(part 1 of 3)
# Autodesk Inventor assembly: Frame 1771926384246
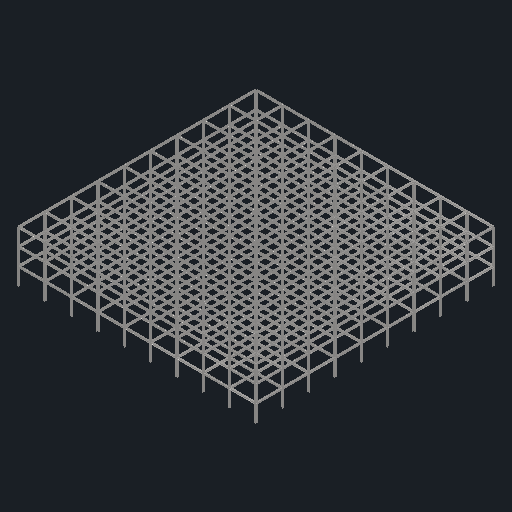
[picture p0: Inventor's stored thumbnail of the model, 512x512]
Saved by Autodesk Inventor 2026.2 (Build 302298010, 298A)
## iProperties
Created: 2026-02-24
Part Number: Frame 1771926384246
Document SubType Name: Assembly
Designer: Admin01
_FrameDoc: Frame Assembly
_Version: 15.0.0
Author: Admin01
## Documents named in this file (842)
- C:\Users\Admin01\Documents\WU15\TRASTRGNN\Inventor\StructureGenerator\Frame\Frame 1771926384246.iam
- C:\Users\Admin01\Documents\WU15\TRASTRGNN\Inventor\StructureGenerator\Frame\Skeleton 1771926384247.ipt
- C:\Users\Admin01\Documents\WU15\TRASTRGNN\Inventor\StructureGenerator\Frame\ANSI UP8 x 30 1771926386924.ipt
- C:\Users\Admin01\Documents\WU15\TRASTRGNN\Inventor\StructureGenerator\Frame\ANSI UP8 x 30 1771926386954.ipt
- C:\Users\Admin01\Documents\WU15\TRASTRGNN\Inventor\StructureGenerator\Frame\ANSI UP8 x 30 1771926386984.ipt
- C:\Users\Admin01\Documents\WU15\TRASTRGNN\Inventor\StructureGenerator\Frame\ANSI UP8 x 30 1771926387014.ipt
- C:\Users\Admin01\Documents\WU15\TRASTRGNN\Inventor\StructureGenerator\Frame\ANSI UP8 x 30 1771926387045.ipt
- C:\Users\Admin01\Documents\WU15\TRASTRGNN\Inventor\StructureGenerator\Frame\ANSI UP8 x 30 1771926387076.ipt
- C:\Users\Admin01\Documents\WU15\TRASTRGNN\Inventor\StructureGenerator\Frame\ANSI UP8 x 30 1771926387107.ipt
- C:\Users\Admin01\Documents\WU15\TRASTRGNN\Inventor\StructureGenerator\Frame\ANSI UP8 x 30 1771926387138.ipt
- C:\Users\Admin01\Documents\WU15\TRASTRGNN\Inventor\StructureGenerator\Frame\ANSI UP8 x 30 1771926387168.ipt
- C:\Users\Admin01\Documents\WU15\TRASTRGNN\Inventor\StructureGenerator\Frame\ANSI UP8 x 30 1771926387199.ipt
- C:\Users\Admin01\Documents\WU15\TRASTRGNN\Inventor\StructureGenerator\Frame\ANSI UP8 x 30 1771926387229.ipt
- C:\Users\Admin01\Documents\WU15\TRASTRGNN\Inventor\StructureGenerator\Frame\ANSI UP8 x 30 1771926387258.ipt
- C:\Users\Admin01\Documents\WU15\TRASTRGNN\Inventor\StructureGenerator\Frame\ANSI UP8 x 30 1771926387288.ipt
- C:\Users\Admin01\Documents\WU15\TRASTRGNN\Inventor\StructureGenerator\Frame\ANSI UP8 x 30 1771926387318.ipt
- C:\Users\Admin01\Documents\WU15\TRASTRGNN\Inventor\StructureGenerator\Frame\ANSI UP8 x 30 1771926387348.ipt
- C:\Users\Admin01\Documents\WU15\TRASTRGNN\Inventor\StructureGenerator\Frame\ANSI UP8 x 30 1771926387378.ipt
- C:\Users\Admin01\Documents\WU15\TRASTRGNN\Inventor\StructureGenerator\Frame\ANSI UP8 x 30 1771926387408.ipt
- C:\Users\Admin01\Documents\WU15\TRASTRGNN\Inventor\StructureGenerator\Frame\ANSI UP8 x 30 1771926387438.ipt
- C:\Users\Admin01\Documents\WU15\TRASTRGNN\Inventor\StructureGenerator\Frame\ANSI UP8 x 30 1771926387467.ipt
- C:\Users\Admin01\Documents\WU15\TRASTRGNN\Inventor\StructureGenerator\Frame\ANSI UP8 x 30 1771926387497.ipt
- C:\Users\Admin01\Documents\WU15\TRASTRGNN\Inventor\StructureGenerator\Frame\ANSI UP8 x 30 1771926387527.ipt
- C:\Users\Admin01\Documents\WU15\TRASTRGNN\Inventor\StructureGenerator\Frame\ANSI UP8 x 30 1771926387557.ipt
- C:\Users\Admin01\Documents\WU15\TRASTRGNN\Inventor\StructureGenerator\Frame\ANSI UP8 x 30 1771926387586.ipt
- C:\Users\Admin01\Documents\WU15\TRASTRGNN\Inventor\StructureGenerator\Frame\ANSI UP8 x 30 1771926387616.ipt
- C:\Users\Admin01\Documents\WU15\TRASTRGNN\Inventor\StructureGenerator\Frame\ANSI UP8 x 30 1771926387646.ipt
- C:\Users\Admin01\Documents\WU15\TRASTRGNN\Inventor\StructureGenerator\Frame\ANSI UP8 x 30 1771926387675.ipt
- C:\Users\Admin01\Documents\WU15\TRASTRGNN\Inventor\StructureGenerator\Frame\ANSI UP8 x 30 1771926387705.ipt
- C:\Users\Admin01\Documents\WU15\TRASTRGNN\Inventor\StructureGenerator\Frame\ANSI UP8 x 30 1771926387735.ipt
- C:\Users\Admin01\Documents\WU15\TRASTRGNN\Inventor\StructureGenerator\Frame\ANSI UP8 x 30 1771926387764.ipt
- C:\Users\Admin01\Documents\WU15\TRASTRGNN\Inventor\StructureGenerator\Frame\ANSI UP8 x 30 1771926387794.ipt
- C:\Users\Admin01\Documents\WU15\TRASTRGNN\Inventor\StructureGenerator\Frame\ANSI UP8 x 30 1771926387824.ipt
- C:\Users\Admin01\Documents\WU15\TRASTRGNN\Inventor\StructureGenerator\Frame\ANSI UP8 x 30 1771926387853.ipt
- C:\Users\Admin01\Documents\WU15\TRASTRGNN\Inventor\StructureGenerator\Frame\ANSI UP8 x 30 1771926387882.ipt
- C:\Users\Admin01\Documents\WU15\TRASTRGNN\Inventor\StructureGenerator\Frame\ANSI UP8 x 30 1771926387912.ipt
- C:\Users\Admin01\Documents\WU15\TRASTRGNN\Inventor\StructureGenerator\Frame\ANSI UP8 x 30 1771926387945.ipt
- C:\Users\Admin01\Documents\WU15\TRASTRGNN\Inventor\StructureGenerator\Frame\ANSI UP8 x 30 1771926387975.ipt
- C:\Users\Admin01\Documents\WU15\TRASTRGNN\Inventor\StructureGenerator\Frame\ANSI UP8 x 30 1771926388005.ipt
- C:\Users\Admin01\Documents\WU15\TRASTRGNN\Inventor\StructureGenerator\Frame\ANSI UP8 x 30 1771926388034.ipt
- C:\Users\Admin01\Documents\WU15\TRASTRGNN\Inventor\StructureGenerator\Frame\ANSI UP8 x 30 1771926388063.ipt
- C:\Users\Admin01\Documents\WU15\TRASTRGNN\Inventor\StructureGenerator\Frame\ANSI UP8 x 30 1771926388093.ipt
- C:\Users\Admin01\Documents\WU15\TRASTRGNN\Inventor\StructureGenerator\Frame\ANSI UP8 x 30 1771926388122.ipt
- C:\Users\Admin01\Documents\WU15\TRASTRGNN\Inventor\StructureGenerator\Frame\ANSI UP8 x 30 1771926388152.ipt
- C:\Users\Admin01\Documents\WU15\TRASTRGNN\Inventor\StructureGenerator\Frame\ANSI UP8 x 30 1771926388182.ipt
- C:\Users\Admin01\Documents\WU15\TRASTRGNN\Inventor\StructureGenerator\Frame\ANSI UP8 x 30 1771926388211.ipt
- C:\Users\Admin01\Documents\WU15\TRASTRGNN\Inventor\StructureGenerator\Frame\ANSI UP8 x 30 1771926388240.ipt
- C:\Users\Admin01\Documents\WU15\TRASTRGNN\Inventor\StructureGenerator\Frame\ANSI UP8 x 30 1771926388269.ipt
- C:\Users\Admin01\Documents\WU15\TRASTRGNN\Inventor\StructureGenerator\Frame\ANSI UP8 x 30 1771926388299.ipt
- C:\Users\Admin01\Documents\WU15\TRASTRGNN\Inventor\StructureGenerator\Frame\ANSI UP8 x 30 1771926388328.ipt
- C:\Users\Admin01\Documents\WU15\TRASTRGNN\Inventor\StructureGenerator\Frame\ANSI UP8 x 30 1771926388357.ipt
- C:\Users\Admin01\Documents\WU15\TRASTRGNN\Inventor\StructureGenerator\Frame\ANSI UP8 x 30 1771926388386.ipt
- C:\Users\Admin01\Documents\WU15\TRASTRGNN\Inventor\StructureGenerator\Frame\ANSI UP8 x 30 1771926388416.ipt
- C:\Users\Admin01\Documents\WU15\TRASTRGNN\Inventor\StructureGenerator\Frame\ANSI UP8 x 30 1771926388446.ipt
- C:\Users\Admin01\Documents\WU15\TRASTRGNN\Inventor\StructureGenerator\Frame\ANSI UP8 x 30 1771926388475.ipt
- C:\Users\Admin01\Documents\WU15\TRASTRGNN\Inventor\StructureGenerator\Frame\ANSI UP8 x 30 1771926388505.ipt
- C:\Users\Admin01\Documents\WU15\TRASTRGNN\Inventor\StructureGenerator\Frame\ANSI UP8 x 30 1771926388535.ipt
- C:\Users\Admin01\Documents\WU15\TRASTRGNN\Inventor\StructureGenerator\Frame\ANSI UP8 x 30 1771926388565.ipt
- C:\Users\Admin01\Documents\WU15\TRASTRGNN\Inventor\StructureGenerator\Frame\ANSI UP8 x 30 1771926388594.ipt
- C:\Users\Admin01\Documents\WU15\TRASTRGNN\Inventor\StructureGenerator\Frame\ANSI UP8 x 30 1771926388624.ipt
- C:\Users\Admin01\Documents\WU15\TRASTRGNN\Inventor\StructureGenerator\Frame\ANSI UP8 x 30 1771926388653.ipt
- C:\Users\Admin01\Documents\WU15\TRASTRGNN\Inventor\StructureGenerator\Frame\ANSI UP8 x 30 1771926388683.ipt
- C:\Users\Admin01\Documents\WU15\TRASTRGNN\Inventor\StructureGenerator\Frame\ANSI UP8 x 30 1771926388713.ipt
- C:\Users\Admin01\Documents\WU15\TRASTRGNN\Inventor\StructureGenerator\Frame\ANSI UP8 x 30 1771926388742.ipt
- C:\Users\Admin01\Documents\WU15\TRASTRGNN\Inventor\StructureGenerator\Frame\ANSI UP8 x 30 1771926388771.ipt
- C:\Users\Admin01\Documents\WU15\TRASTRGNN\Inventor\StructureGenerator\Frame\ANSI UP8 x 30 1771926388800.ipt
- C:\Users\Admin01\Documents\WU15\TRASTRGNN\Inventor\StructureGenerator\Frame\ANSI UP8 x 30 1771926388830.ipt
- C:\Users\Admin01\Documents\WU15\TRASTRGNN\Inventor\StructureGenerator\Frame\ANSI UP8 x 30 1771926388859.ipt
- C:\Users\Admin01\Documents\WU15\TRASTRGNN\Inventor\StructureGenerator\Frame\ANSI UP8 x 30 1771926388888.ipt
- C:\Users\Admin01\Documents\WU15\TRASTRGNN\Inventor\StructureGenerator\Frame\ANSI UP8 x 30 1771926388918.ipt
- C:\Users\Admin01\Documents\WU15\TRASTRGNN\Inventor\StructureGenerator\Frame\ANSI UP8 x 30 1771926388947.ipt
- C:\Users\Admin01\Documents\WU15\TRASTRGNN\Inventor\StructureGenerator\Frame\ANSI UP8 x 30 1771926388977.ipt
- C:\Users\Admin01\Documents\WU15\TRASTRGNN\Inventor\StructureGenerator\Frame\ANSI UP8 x 30 1771926389006.ipt
- C:\Users\Admin01\Documents\WU15\TRASTRGNN\Inventor\StructureGenerator\Frame\ANSI UP8 x 30 1771926389039.ipt
- C:\Users\Admin01\Documents\WU15\TRASTRGNN\Inventor\StructureGenerator\Frame\ANSI UP8 x 30 1771926389068.ipt
- C:\Users\Admin01\Documents\WU15\TRASTRGNN\Inventor\StructureGenerator\Frame\ANSI UP8 x 30 1771926389098.ipt
- C:\Users\Admin01\Documents\WU15\TRASTRGNN\Inventor\StructureGenerator\Frame\ANSI UP8 x 30 1771926389128.ipt
- C:\Users\Admin01\Documents\WU15\TRASTRGNN\Inventor\StructureGenerator\Frame\ANSI UP8 x 30 1771926389158.ipt
- C:\Users\Admin01\Documents\WU15\TRASTRGNN\Inventor\StructureGenerator\Frame\ANSI UP8 x 30 1771926389187.ipt
- C:\Users\Admin01\Documents\WU15\TRASTRGNN\Inventor\StructureGenerator\Frame\ANSI UP8 x 30 1771926389216.ipt
- C:\Users\Admin01\Documents\WU15\TRASTRGNN\Inventor\StructureGenerator\Frame\ANSI UP8 x 30 1771926389245.ipt
- C:\Users\Admin01\Documents\WU15\TRASTRGNN\Inventor\StructureGenerator\Frame\ANSI UP8 x 30 1771926389274.ipt
- C:\Users\Admin01\Documents\WU15\TRASTRGNN\Inventor\StructureGenerator\Frame\ANSI UP8 x 30 1771926389303.ipt
- C:\Users\Admin01\Documents\WU15\TRASTRGNN\Inventor\StructureGenerator\Frame\ANSI UP8 x 30 1771926389333.ipt
- C:\Users\Admin01\Documents\WU15\TRASTRGNN\Inventor\StructureGenerator\Frame\ANSI UP8 x 30 1771926389362.ipt
- C:\Users\Admin01\Documents\WU15\TRASTRGNN\Inventor\StructureGenerator\Frame\ANSI UP8 x 30 1771926389391.ipt
- C:\Users\Admin01\Documents\WU15\TRASTRGNN\Inventor\StructureGenerator\Frame\ANSI UP8 x 30 1771926389420.ipt
- C:\Users\Admin01\Documents\WU15\TRASTRGNN\Inventor\StructureGenerator\Frame\ANSI UP8 x 30 1771926389450.ipt
- C:\Users\Admin01\Documents\WU15\TRASTRGNN\Inventor\StructureGenerator\Frame\ANSI UP8 x 30 1771926389479.ipt
- C:\Users\Admin01\Documents\WU15\TRASTRGNN\Inventor\StructureGenerator\Frame\ANSI UP8 x 30 1771926389515.ipt
- C:\Users\Admin01\Documents\WU15\TRASTRGNN\Inventor\StructureGenerator\Frame\ANSI UP8 x 30 1771926389551.ipt
- C:\Users\Admin01\Documents\WU15\TRASTRGNN\Inventor\StructureGenerator\Frame\ANSI UP8 x 30 1771926389587.ipt
- C:\Users\Admin01\Documents\WU15\TRASTRGNN\Inventor\StructureGenerator\Frame\ANSI UP8 x 30 1771926389625.ipt
- C:\Users\Admin01\Documents\WU15\TRASTRGNN\Inventor\StructureGenerator\Frame\ANSI UP8 x 30 1771926389656.ipt
- C:\Users\Admin01\Documents\WU15\TRASTRGNN\Inventor\StructureGenerator\Frame\ANSI UP8 x 30 1771926389685.ipt
- C:\Users\Admin01\Documents\WU15\TRASTRGNN\Inventor\StructureGenerator\Frame\ANSI UP8 x 30 1771926389715.ipt
- C:\Users\Admin01\Documents\WU15\TRASTRGNN\Inventor\StructureGenerator\Frame\ANSI UP8 x 30 1771926389744.ipt
- C:\Users\Admin01\Documents\WU15\TRASTRGNN\Inventor\StructureGenerator\Frame\ANSI UP8 x 30 1771926389773.ipt
- C:\Users\Admin01\Documents\WU15\TRASTRGNN\Inventor\StructureGenerator\Frame\ANSI UP8 x 30 1771926389802.ipt
- C:\Users\Admin01\Documents\WU15\TRASTRGNN\Inventor\StructureGenerator\Frame\ANSI UP8 x 30 1771926389831.ipt
- C:\Users\Admin01\Documents\WU15\TRASTRGNN\Inventor\StructureGenerator\Frame\ANSI UP8 x 30 1771926389860.ipt
- C:\Users\Admin01\Documents\WU15\TRASTRGNN\Inventor\StructureGenerator\Frame\ANSI UP8 x 30 1771926389889.ipt
- C:\Users\Admin01\Documents\WU15\TRASTRGNN\Inventor\StructureGenerator\Frame\ANSI UP8 x 30 1771926389918.ipt
- C:\Users\Admin01\Documents\WU15\TRASTRGNN\Inventor\StructureGenerator\Frame\ANSI UP8 x 30 1771926389947.ipt
- C:\Users\Admin01\Documents\WU15\TRASTRGNN\Inventor\StructureGenerator\Frame\ANSI UP8 x 30 1771926389976.ipt
- C:\Users\Admin01\Documents\WU15\TRASTRGNN\Inventor\StructureGenerator\Frame\ANSI UP8 x 30 1771926390006.ipt
- C:\Users\Admin01\Documents\WU15\TRASTRGNN\Inventor\StructureGenerator\Frame\ANSI UP8 x 30 1771926390034.ipt
- C:\Users\Admin01\Documents\WU15\TRASTRGNN\Inventor\StructureGenerator\Frame\ANSI UP8 x 30 1771926390064.ipt
- C:\Users\Admin01\Documents\WU15\TRASTRGNN\Inventor\StructureGenerator\Frame\ANSI UP8 x 30 1771926390093.ipt
- C:\Users\Admin01\Documents\WU15\TRASTRGNN\Inventor\StructureGenerator\Frame\ANSI UP8 x 30 1771926390122.ipt
- C:\Users\Admin01\Documents\WU15\TRASTRGNN\Inventor\StructureGenerator\Frame\ANSI UP8 x 30 1771926390154.ipt
- C:\Users\Admin01\Documents\WU15\TRASTRGNN\Inventor\StructureGenerator\Frame\ANSI UP8 x 30 1771926390184.ipt
- C:\Users\Admin01\Documents\WU15\TRASTRGNN\Inventor\StructureGenerator\Frame\ANSI UP8 x 30 1771926390213.ipt
- C:\Users\Admin01\Documents\WU15\TRASTRGNN\Inventor\StructureGenerator\Frame\ANSI UP8 x 30 1771926390246.ipt
- C:\Users\Admin01\Documents\WU15\TRASTRGNN\Inventor\StructureGenerator\Frame\ANSI UP8 x 30 1771926390275.ipt
- C:\Users\Admin01\Documents\WU15\TRASTRGNN\Inventor\StructureGenerator\Frame\ANSI UP8 x 30 1771926390304.ipt
- C:\Users\Admin01\Documents\WU15\TRASTRGNN\Inventor\StructureGenerator\Frame\ANSI UP8 x 30 1771926390333.ipt
- C:\Users\Admin01\Documents\WU15\TRASTRGNN\Inventor\StructureGenerator\Frame\ANSI UP8 x 30 1771926390362.ipt
- C:\Users\Admin01\Documents\WU15\TRASTRGNN\Inventor\StructureGenerator\Frame\ANSI UP8 x 30 1771926390391.ipt
- C:\Users\Admin01\Documents\WU15\TRASTRGNN\Inventor\StructureGenerator\Frame\ANSI UP8 x 30 1771926390421.ipt
- C:\Users\Admin01\Documents\WU15\TRASTRGNN\Inventor\StructureGenerator\Frame\ANSI UP8 x 30 1771926390450.ipt
- C:\Users\Admin01\Documents\WU15\TRASTRGNN\Inventor\StructureGenerator\Frame\ANSI UP8 x 30 1771926390480.ipt
- C:\Users\Admin01\Documents\WU15\TRASTRGNN\Inventor\StructureGenerator\Frame\ANSI UP8 x 30 1771926390509.ipt
- C:\Users\Admin01\Documents\WU15\TRASTRGNN\Inventor\StructureGenerator\Frame\ANSI UP8 x 30 1771926390539.ipt
- C:\Users\Admin01\Documents\WU15\TRASTRGNN\Inventor\StructureGenerator\Frame\ANSI UP8 x 30 1771926390569.ipt
- C:\Users\Admin01\Documents\WU15\TRASTRGNN\Inventor\StructureGenerator\Frame\ANSI UP8 x 30 1771926390598.ipt
- C:\Users\Admin01\Documents\WU15\TRASTRGNN\Inventor\StructureGenerator\Frame\ANSI UP8 x 30 1771926390628.ipt
- C:\Users\Admin01\Documents\WU15\TRASTRGNN\Inventor\StructureGenerator\Frame\ANSI UP8 x 30 1771926390658.ipt
- C:\Users\Admin01\Documents\WU15\TRASTRGNN\Inventor\StructureGenerator\Frame\ANSI UP8 x 30 1771926390687.ipt
- C:\Users\Admin01\Documents\WU15\TRASTRGNN\Inventor\StructureGenerator\Frame\ANSI UP8 x 30 1771926390716.ipt
- C:\Users\Admin01\Documents\WU15\TRASTRGNN\Inventor\StructureGenerator\Frame\ANSI UP8 x 30 1771926390746.ipt
- C:\Users\Admin01\Documents\WU15\TRASTRGNN\Inventor\StructureGenerator\Frame\ANSI UP8 x 30 1771926390776.ipt
- C:\Users\Admin01\Documents\WU15\TRASTRGNN\Inventor\StructureGenerator\Frame\ANSI UP8 x 30 1771926390806.ipt
- C:\Users\Admin01\Documents\WU15\TRASTRGNN\Inventor\StructureGenerator\Frame\ANSI UP8 x 30 1771926390836.ipt
- C:\Users\Admin01\Documents\WU15\TRASTRGNN\Inventor\StructureGenerator\Frame\ANSI UP8 x 30 1771926390865.ipt
- C:\Users\Admin01\Documents\WU15\TRASTRGNN\Inventor\StructureGenerator\Frame\ANSI UP8 x 30 1771926390894.ipt
- C:\Users\Admin01\Documents\WU15\TRASTRGNN\Inventor\StructureGenerator\Frame\ANSI UP8 x 30 1771926390924.ipt
- C:\Users\Admin01\Documents\WU15\TRASTRGNN\Inventor\StructureGenerator\Frame\ANSI UP8 x 30 1771926390953.ipt
- C:\Users\Admin01\Documents\WU15\TRASTRGNN\Inventor\StructureGenerator\Frame\ANSI UP8 x 30 1771926390983.ipt
- C:\Users\Admin01\Documents\WU15\TRASTRGNN\Inventor\StructureGenerator\Frame\ANSI UP8 x 30 1771926391012.ipt
- C:\Users\Admin01\Documents\WU15\TRASTRGNN\Inventor\StructureGenerator\Frame\ANSI UP8 x 30 1771926391042.ipt
- C:\Users\Admin01\Documents\WU15\TRASTRGNN\Inventor\StructureGenerator\Frame\ANSI UP8 x 30 1771926391071.ipt
- C:\Users\Admin01\Documents\WU15\TRASTRGNN\Inventor\StructureGenerator\Frame\ANSI UP8 x 30 1771926391102.ipt
- C:\Users\Admin01\Documents\WU15\TRASTRGNN\Inventor\StructureGenerator\Frame\ANSI UP8 x 30 1771926391131.ipt
- C:\Users\Admin01\Documents\WU15\TRASTRGNN\Inventor\StructureGenerator\Frame\ANSI UP8 x 30 1771926391160.ipt
- C:\Users\Admin01\Documents\WU15\TRASTRGNN\Inventor\StructureGenerator\Frame\ANSI UP8 x 30 1771926391190.ipt
- C:\Users\Admin01\Documents\WU15\TRASTRGNN\Inventor\StructureGenerator\Frame\ANSI UP8 x 30 1771926391219.ipt
- C:\Users\Admin01\Documents\WU15\TRASTRGNN\Inventor\StructureGenerator\Frame\ANSI UP8 x 30 1771926391252.ipt
- C:\Users\Admin01\Documents\WU15\TRASTRGNN\Inventor\StructureGenerator\Frame\ANSI UP8 x 30 1771926391282.ipt
- C:\Users\Admin01\Documents\WU15\TRASTRGNN\Inventor\StructureGenerator\Frame\ANSI UP8 x 30 1771926391311.ipt
- C:\Users\Admin01\Documents\WU15\TRASTRGNN\Inventor\StructureGenerator\Frame\ANSI UP8 x 30 1771926391340.ipt
- C:\Users\Admin01\Documents\WU15\TRASTRGNN\Inventor\StructureGenerator\Frame\ANSI UP8 x 30 1771926391369.ipt
- C:\Users\Admin01\Documents\WU15\TRASTRGNN\Inventor\StructureGenerator\Frame\ANSI UP8 x 30 1771926391399.ipt
- C:\Users\Admin01\Documents\WU15\TRASTRGNN\Inventor\StructureGenerator\Frame\ANSI UP8 x 30 1771926391428.ipt
- C:\Users\Admin01\Documents\WU15\TRASTRGNN\Inventor\StructureGenerator\Frame\ANSI UP8 x 30 1771926391457.ipt
- C:\Users\Admin01\Documents\WU15\TRASTRGNN\Inventor\StructureGenerator\Frame\ANSI UP8 x 30 1771926391486.ipt
- C:\Users\Admin01\Documents\WU15\TRASTRGNN\Inventor\StructureGenerator\Frame\ANSI UP8 x 30 1771926391515.ipt
- C:\Users\Admin01\Documents\WU15\TRASTRGNN\Inventor\StructureGenerator\Frame\ANSI UP8 x 30 1771926391549.ipt
- C:\Users\Admin01\Documents\WU15\TRASTRGNN\Inventor\StructureGenerator\Frame\ANSI UP8 x 30 1771926391578.ipt
- C:\Users\Admin01\Documents\WU15\TRASTRGNN\Inventor\StructureGenerator\Frame\ANSI UP8 x 30 1771926391608.ipt
- C:\Users\Admin01\Documents\WU15\TRASTRGNN\Inventor\StructureGenerator\Frame\ANSI UP8 x 30 1771926391637.ipt
- C:\Users\Admin01\Documents\WU15\TRASTRGNN\Inventor\StructureGenerator\Frame\ANSI UP8 x 30 1771926391667.ipt
- C:\Users\Admin01\Documents\WU15\TRASTRGNN\Inventor\StructureGenerator\Frame\ANSI UP8 x 30 1771926391696.ipt
- C:\Users\Admin01\Documents\WU15\TRASTRGNN\Inventor\StructureGenerator\Frame\ANSI UP8 x 30 1771926391725.ipt
- C:\Users\Admin01\Documents\WU15\TRASTRGNN\Inventor\StructureGenerator\Frame\ANSI UP8 x 30 1771926391754.ipt
- C:\Users\Admin01\Documents\WU15\TRASTRGNN\Inventor\StructureGenerator\Frame\ANSI UP8 x 30 1771926391784.ipt
- C:\Users\Admin01\Documents\WU15\TRASTRGNN\Inventor\StructureGenerator\Frame\ANSI UP8 x 30 1771926391813.ipt
- C:\Users\Admin01\Documents\WU15\TRASTRGNN\Inventor\StructureGenerator\Frame\ANSI UP8 x 30 1771926391842.ipt
- C:\Users\Admin01\Documents\WU15\TRASTRGNN\Inventor\StructureGenerator\Frame\ANSI UP8 x 30 1771926391871.ipt
- C:\Users\Admin01\Documents\WU15\TRASTRGNN\Inventor\StructureGenerator\Frame\ANSI UP8 x 30 1771926391900.ipt
- C:\Users\Admin01\Documents\WU15\TRASTRGNN\Inventor\StructureGenerator\Frame\ANSI UP8 x 30 1771926391930.ipt
- C:\Users\Admin01\Documents\WU15\TRASTRGNN\Inventor\StructureGenerator\Frame\ANSI UP8 x 30 1771926391960.ipt
- C:\Users\Admin01\Documents\WU15\TRASTRGNN\Inventor\StructureGenerator\Frame\ANSI UP8 x 30 1771926391990.ipt
- C:\Users\Admin01\Documents\WU15\TRASTRGNN\Inventor\StructureGenerator\Frame\ANSI UP8 x 30 1771926392019.ipt
- C:\Users\Admin01\Documents\WU15\TRASTRGNN\Inventor\StructureGenerator\Frame\ANSI UP8 x 30 1771926392048.ipt
- C:\Users\Admin01\Documents\WU15\TRASTRGNN\Inventor\StructureGenerator\Frame\ANSI UP8 x 30 1771926392077.ipt
- C:\Users\Admin01\Documents\WU15\TRASTRGNN\Inventor\StructureGenerator\Frame\ANSI UP8 x 30 1771926392107.ipt
- C:\Users\Admin01\Documents\WU15\TRASTRGNN\Inventor\StructureGenerator\Frame\ANSI UP8 x 30 1771926392136.ipt
- C:\Users\Admin01\Documents\WU15\TRASTRGNN\Inventor\StructureGenerator\Frame\ANSI UP8 x 30 1771926392166.ipt
- C:\Users\Admin01\Documents\WU15\TRASTRGNN\Inventor\StructureGenerator\Frame\ANSI UP8 x 30 1771926392195.ipt
- C:\Users\Admin01\Documents\WU15\TRASTRGNN\Inventor\StructureGenerator\Frame\ANSI UP8 x 30 1771926392224.ipt
- C:\Users\Admin01\Documents\WU15\TRASTRGNN\Inventor\StructureGenerator\Frame\ANSI UP8 x 30 1771926392253.ipt
- C:\Users\Admin01\Documents\WU15\TRASTRGNN\Inventor\StructureGenerator\Frame\ANSI UP8 x 30 1771926392282.ipt
- C:\Users\Admin01\Documents\WU15\TRASTRGNN\Inventor\StructureGenerator\Frame\ANSI UP8 x 30 1771926392311.ipt
- C:\Users\Admin01\Documents\WU15\TRASTRGNN\Inventor\StructureGenerator\Frame\ANSI UP8 x 30 1771926392344.ipt
- C:\Users\Admin01\Documents\WU15\TRASTRGNN\Inventor\StructureGenerator\Frame\ANSI UP8 x 30 1771926392373.ipt
- C:\Users\Admin01\Documents\WU15\TRASTRGNN\Inventor\StructureGenerator\Frame\ANSI UP8 x 30 1771926392402.ipt
- C:\Users\Admin01\Documents\WU15\TRASTRGNN\Inventor\StructureGenerator\Frame\ANSI UP8 x 30 1771926392432.ipt
- C:\Users\Admin01\Documents\WU15\TRASTRGNN\Inventor\StructureGenerator\Frame\ANSI UP8 x 30 1771926392461.ipt
- C:\Users\Admin01\Documents\WU15\TRASTRGNN\Inventor\StructureGenerator\Frame\ANSI UP8 x 30 1771926392490.ipt
- C:\Users\Admin01\Documents\WU15\TRASTRGNN\Inventor\StructureGenerator\Frame\ANSI UP8 x 30 1771926392520.ipt
- C:\Users\Admin01\Documents\WU15\TRASTRGNN\Inventor\StructureGenerator\Frame\ANSI UP8 x 30 1771926392549.ipt
- C:\Users\Admin01\Documents\WU15\TRASTRGNN\Inventor\StructureGenerator\Frame\ANSI UP8 x 30 1771926392578.ipt
- C:\Users\Admin01\Documents\WU15\TRASTRGNN\Inventor\StructureGenerator\Frame\ANSI UP8 x 30 1771926392607.ipt
- C:\Users\Admin01\Documents\WU15\TRASTRGNN\Inventor\StructureGenerator\Frame\ANSI UP8 x 30 1771926392637.ipt
- C:\Users\Admin01\Documents\WU15\TRASTRGNN\Inventor\StructureGenerator\Frame\ANSI UP8 x 30 1771926392667.ipt
- C:\Users\Admin01\Documents\WU15\TRASTRGNN\Inventor\StructureGenerator\Frame\ANSI UP8 x 30 1771926392696.ipt
- C:\Users\Admin01\Documents\WU15\TRASTRGNN\Inventor\StructureGenerator\Frame\ANSI UP8 x 30 1771926392725.ipt
- C:\Users\Admin01\Documents\WU15\TRASTRGNN\Inventor\StructureGenerator\Frame\ANSI UP8 x 30 1771926392755.ipt
- C:\Users\Admin01\Documents\WU15\TRASTRGNN\Inventor\StructureGenerator\Frame\ANSI UP8 x 30 1771926392784.ipt
- C:\Users\Admin01\Documents\WU15\TRASTRGNN\Inventor\StructureGenerator\Frame\ANSI UP8 x 30 1771926392813.ipt
- C:\Users\Admin01\Documents\WU15\TRASTRGNN\Inventor\StructureGenerator\Frame\ANSI UP8 x 30 1771926392842.ipt
- C:\Users\Admin01\Documents\WU15\TRASTRGNN\Inventor\StructureGenerator\Frame\ANSI UP8 x 30 1771926392872.ipt
- C:\Users\Admin01\Documents\WU15\TRASTRGNN\Inventor\StructureGenerator\Frame\ANSI UP8 x 30 1771926392901.ipt
- C:\Users\Admin01\Documents\WU15\TRASTRGNN\Inventor\StructureGenerator\Frame\ANSI UP8 x 30 1771926392930.ipt
- C:\Users\Admin01\Documents\WU15\TRASTRGNN\Inventor\StructureGenerator\Frame\ANSI UP8 x 30 1771926392960.ipt
- C:\Users\Admin01\Documents\WU15\TRASTRGNN\Inventor\StructureGenerator\Frame\ANSI UP8 x 30 1771926392989.ipt
- C:\Users\Admin01\Documents\WU15\TRASTRGNN\Inventor\StructureGenerator\Frame\ANSI UP8 x 30 1771926393018.ipt
- C:\Users\Admin01\Documents\WU15\TRASTRGNN\Inventor\StructureGenerator\Frame\ANSI UP8 x 30 1771926393048.ipt
- C:\Users\Admin01\Documents\WU15\TRASTRGNN\Inventor\StructureGenerator\Frame\ANSI UP8 x 30 1771926393077.ipt
- C:\Users\Admin01\Documents\WU15\TRASTRGNN\Inventor\StructureGenerator\Frame\ANSI UP8 x 30 1771926393106.ipt
- C:\Users\Admin01\Documents\WU15\TRASTRGNN\Inventor\StructureGenerator\Frame\ANSI UP8 x 30 1771926393136.ipt
- C:\Users\Admin01\Documents\WU15\TRASTRGNN\Inventor\StructureGenerator\Frame\ANSI UP8 x 30 1771926393166.ipt
- C:\Users\Admin01\Documents\WU15\TRASTRGNN\Inventor\StructureGenerator\Frame\ANSI UP8 x 30 1771926393196.ipt
- C:\Users\Admin01\Documents\WU15\TRASTRGNN\Inventor\StructureGenerator\Frame\ANSI UP8 x 30 1771926393225.ipt
- C:\Users\Admin01\Documents\WU15\TRASTRGNN\Inventor\StructureGenerator\Frame\ANSI UP8 x 30 1771926393255.ipt
- C:\Users\Admin01\Documents\WU15\TRASTRGNN\Inventor\StructureGenerator\Frame\ANSI UP8 x 30 1771926393284.ipt
- C:\Users\Admin01\Documents\WU15\TRASTRGNN\Inventor\StructureGenerator\Frame\ANSI UP8 x 30 1771926393313.ipt
- C:\Users\Admin01\Documents\WU15\TRASTRGNN\Inventor\StructureGenerator\Frame\ANSI UP8 x 30 1771926393342.ipt
- C:\Users\Admin01\Documents\WU15\TRASTRGNN\Inventor\StructureGenerator\Frame\ANSI UP8 x 30 1771926393371.ipt
- C:\Users\Admin01\Documents\WU15\TRASTRGNN\Inventor\StructureGenerator\Frame\ANSI UP8 x 30 1771926393400.ipt
- C:\Users\Admin01\Documents\WU15\TRASTRGNN\Inventor\StructureGenerator\Frame\ANSI UP8 x 30 1771926393451.ipt
- C:\Users\Admin01\Documents\WU15\TRASTRGNN\Inventor\StructureGenerator\Frame\ANSI UP8 x 30 1771926393482.ipt
- C:\Users\Admin01\Documents\WU15\TRASTRGNN\Inventor\StructureGenerator\Frame\ANSI UP8 x 30 1771926393513.ipt
- C:\Users\Admin01\Documents\WU15\TRASTRGNN\Inventor\StructureGenerator\Frame\ANSI UP8 x 30 1771926393543.ipt
- C:\Users\Admin01\Documents\WU15\TRASTRGNN\Inventor\StructureGenerator\Frame\ANSI UP8 x 30 1771926393573.ipt
- C:\Users\Admin01\Documents\WU15\TRASTRGNN\Inventor\StructureGenerator\Frame\ANSI UP8 x 30 1771926393603.ipt
- C:\Users\Admin01\Documents\WU15\TRASTRGNN\Inventor\StructureGenerator\Frame\ANSI UP8 x 30 1771926393633.ipt
- C:\Users\Admin01\Documents\WU15\TRASTRGNN\Inventor\StructureGenerator\Frame\ANSI UP8 x 30 1771926393663.ipt
- C:\Users\Admin01\Documents\WU15\TRASTRGNN\Inventor\StructureGenerator\Frame\ANSI UP8 x 30 1771926393693.ipt
- C:\Users\Admin01\Documents\WU15\TRASTRGNN\Inventor\StructureGenerator\Frame\ANSI UP8 x 30 1771926393723.ipt
- C:\Users\Admin01\Documents\WU15\TRASTRGNN\Inventor\StructureGenerator\Frame\ANSI UP8 x 30 1771926393758.ipt
- C:\Users\Admin01\Documents\WU15\TRASTRGNN\Inventor\StructureGenerator\Frame\ANSI UP8 x 30 1771926393788.ipt
- C:\Users\Admin01\Documents\WU15\TRASTRGNN\Inventor\StructureGenerator\Frame\ANSI UP8 x 30 1771926393817.ipt
- C:\Users\Admin01\Documents\WU15\TRASTRGNN\Inventor\StructureGenerator\Frame\ANSI UP8 x 30 1771926393846.ipt
- C:\Users\Admin01\Documents\WU15\TRASTRGNN\Inventor\StructureGenerator\Frame\ANSI UP8 x 30 1771926393875.ipt
- C:\Users\Admin01\Documents\WU15\TRASTRGNN\Inventor\StructureGenerator\Frame\ANSI UP8 x 30 1771926393904.ipt
- C:\Users\Admin01\Documents\WU15\TRASTRGNN\Inventor\StructureGenerator\Frame\ANSI UP8 x 30 1771926393933.ipt
- C:\Users\Admin01\Documents\WU15\TRASTRGNN\Inventor\StructureGenerator\Frame\ANSI UP8 x 30 1771926393963.ipt
- C:\Users\Admin01\Documents\WU15\TRASTRGNN\Inventor\StructureGenerator\Frame\ANSI UP8 x 30 1771926393992.ipt
- C:\Users\Admin01\Documents\WU15\TRASTRGNN\Inventor\StructureGenerator\Frame\ANSI UP8 x 30 1771926394021.ipt
- C:\Users\Admin01\Documents\WU15\TRASTRGNN\Inventor\StructureGenerator\Frame\ANSI UP8 x 30 1771926394050.ipt
- C:\Users\Admin01\Documents\WU15\TRASTRGNN\Inventor\StructureGenerator\Frame\ANSI UP8 x 30 1771926394079.ipt
- C:\Users\Admin01\Documents\WU15\TRASTRGNN\Inventor\StructureGenerator\Frame\ANSI UP8 x 30 1771926394108.ipt
- C:\Users\Admin01\Documents\WU15\TRASTRGNN\Inventor\StructureGenerator\Frame\ANSI UP8 x 30 1771926394137.ipt
- C:\Users\Admin01\Documents\WU15\TRASTRGNN\Inventor\StructureGenerator\Frame\ANSI UP8 x 30 1771926394169.ipt
- C:\Users\Admin01\Documents\WU15\TRASTRGNN\Inventor\StructureGenerator\Frame\ANSI UP8 x 30 1771926394198.ipt
- C:\Users\Admin01\Documents\WU15\TRASTRGNN\Inventor\StructureGenerator\Frame\ANSI UP8 x 30 1771926394228.ipt
- C:\Users\Admin01\Documents\WU15\TRASTRGNN\Inventor\StructureGenerator\Frame\ANSI UP8 x 30 1771926394257.ipt
- C:\Users\Admin01\Documents\WU15\TRASTRGNN\Inventor\StructureGenerator\Frame\ANSI UP8 x 30 1771926394286.ipt
- C:\Users\Admin01\Documents\WU15\TRASTRGNN\Inventor\StructureGenerator\Frame\ANSI UP8 x 30 1771926394316.ipt
- C:\Users\Admin01\Documents\WU15\TRASTRGNN\Inventor\StructureGenerator\Frame\ANSI UP8 x 30 1771926394345.ipt
- C:\Users\Admin01\Documents\WU15\TRASTRGNN\Inventor\StructureGenerator\Frame\ANSI UP8 x 30 1771926394374.ipt
- C:\Users\Admin01\Documents\WU15\TRASTRGNN\Inventor\StructureGenerator\Frame\ANSI UP8 x 30 1771926394404.ipt
- C:\Users\Admin01\Documents\WU15\TRASTRGNN\Inventor\StructureGenerator\Frame\ANSI UP8 x 30 1771926394433.ipt
- C:\Users\Admin01\Documents\WU15\TRASTRGNN\Inventor\StructureGenerator\Frame\ANSI UP8 x 30 1771926394462.ipt
- C:\Users\Admin01\Documents\WU15\TRASTRGNN\Inventor\StructureGenerator\Frame\ANSI UP8 x 30 1771926394492.ipt
- C:\Users\Admin01\Documents\WU15\TRASTRGNN\Inventor\StructureGenerator\Frame\ANSI UP8 x 30 1771926394521.ipt
- C:\Users\Admin01\Documents\WU15\TRASTRGNN\Inventor\StructureGenerator\Frame\ANSI UP8 x 30 1771926394553.ipt
- C:\Users\Admin01\Documents\WU15\TRASTRGNN\Inventor\StructureGenerator\Frame\ANSI UP8 x 30 1771926394582.ipt
- C:\Users\Admin01\Documents\WU15\TRASTRGNN\Inventor\StructureGenerator\Frame\ANSI UP8 x 30 1771926394611.ipt
- C:\Users\Admin01\Documents\WU15\TRASTRGNN\Inventor\StructureGenerator\Frame\ANSI UP8 x 30 1771926394640.ipt
- C:\Users\Admin01\Documents\WU15\TRASTRGNN\Inventor\StructureGenerator\Frame\ANSI UP8 x 30 1771926394669.ipt
- C:\Users\Admin01\Documents\WU15\TRASTRGNN\Inventor\StructureGenerator\Frame\ANSI UP8 x 30 1771926394699.ipt
- C:\Users\Admin01\Documents\WU15\TRASTRGNN\Inventor\StructureGenerator\Frame\ANSI UP8 x 30 1771926394728.ipt
- C:\Users\Admin01\Documents\WU15\TRASTRGNN\Inventor\StructureGenerator\Frame\ANSI UP8 x 30 1771926394757.ipt
- C:\Users\Admin01\Documents\WU15\TRASTRGNN\Inventor\StructureGenerator\Frame\ANSI UP8 x 30 1771926394786.ipt
- C:\Users\Admin01\Documents\WU15\TRASTRGNN\Inventor\StructureGenerator\Frame\ANSI UP8 x 30 1771926394815.ipt
- C:\Users\Admin01\Documents\WU15\TRASTRGNN\Inventor\StructureGenerator\Frame\ANSI UP8 x 30 1771926394844.ipt
- C:\Users\Admin01\Documents\WU15\TRASTRGNN\Inventor\StructureGenerator\Frame\ANSI UP8 x 30 1771926394873.ipt
- C:\Users\Admin01\Documents\WU15\TRASTRGNN\Inventor\StructureGenerator\Frame\ANSI UP8 x 30 1771926394903.ipt
- C:\Users\Admin01\Documents\WU15\TRASTRGNN\Inventor\StructureGenerator\Frame\ANSI UP8 x 30 1771926394932.ipt
- C:\Users\Admin01\Documents\WU15\TRASTRGNN\Inventor\StructureGenerator\Frame\ANSI UP8 x 30 1771926394962.ipt
- C:\Users\Admin01\Documents\WU15\TRASTRGNN\Inventor\StructureGenerator\Frame\ANSI UP8 x 30 1771926394991.ipt
- C:\Users\Admin01\Documents\WU15\TRASTRGNN\Inventor\StructureGenerator\Frame\ANSI UP8 x 30 1771926395021.ipt
- C:\Users\Admin01\Documents\WU15\TRASTRGNN\Inventor\StructureGenerator\Frame\ANSI UP8 x 30 1771926395051.ipt
- C:\Users\Admin01\Documents\WU15\TRASTRGNN\Inventor\StructureGenerator\Frame\ANSI UP8 x 30 1771926395080.ipt
- C:\Users\Admin01\Documents\WU15\TRASTRGNN\Inventor\StructureGenerator\Frame\ANSI UP8 x 30 1771926395109.ipt
- C:\Users\Admin01\Documents\WU15\TRASTRGNN\Inventor\StructureGenerator\Frame\ANSI UP8 x 30 1771926395139.ipt
- C:\Users\Admin01\Documents\WU15\TRASTRGNN\Inventor\StructureGenerator\Frame\ANSI UP8 x 30 1771926395168.ipt
- C:\Users\Admin01\Documents\WU15\TRASTRGNN\Inventor\StructureGenerator\Frame\ANSI UP8 x 30 1771926395197.ipt
- C:\Users\Admin01\Documents\WU15\TRASTRGNN\Inventor\StructureGenerator\Frame\ANSI UP8 x 30 1771926395227.ipt
- C:\Users\Admin01\Documents\WU15\TRASTRGNN\Inventor\StructureGenerator\Frame\ANSI UP8 x 30 1771926395256.ipt
- C:\Users\Admin01\Documents\WU15\TRASTRGNN\Inventor\StructureGenerator\Frame\ANSI UP8 x 30 1771926395285.ipt
- C:\Users\Admin01\Documents\WU15\TRASTRGNN\Inventor\StructureGenerator\Frame\ANSI UP8 x 30 1771926395315.ipt
- C:\Users\Admin01\Documents\WU15\TRASTRGNN\Inventor\StructureGenerator\Frame\ANSI UP8 x 30 1771926395344.ipt
- C:\Users\Admin01\Documents\WU15\TRASTRGNN\Inventor\StructureGenerator\Frame\ANSI UP8 x 30 1771926395373.ipt
- C:\Users\Admin01\Documents\WU15\TRASTRGNN\Inventor\StructureGenerator\Frame\ANSI UP8 x 30 1771926395402.ipt
- C:\Users\Admin01\Documents\WU15\TRASTRGNN\Inventor\StructureGenerator\Frame\ANSI UP8 x 30 1771926395431.ipt
- C:\Users\Admin01\Documents\WU15\TRASTRGNN\Inventor\StructureGenerator\Frame\ANSI UP8 x 30 1771926395460.ipt
- C:\Users\Admin01\Documents\WU15\TRASTRGNN\Inventor\StructureGenerator\Frame\ANSI UP8 x 30 1771926395489.ipt
- C:\Users\Admin01\Documents\WU15\TRASTRGNN\Inventor\StructureGenerator\Frame\ANSI UP8 x 30 1771926395518.ipt
- C:\Users\Admin01\Documents\WU15\TRASTRGNN\Inventor\StructureGenerator\Frame\ANSI UP8 x 30 1771926395548.ipt
- C:\Users\Admin01\Documents\WU15\TRASTRGNN\Inventor\StructureGenerator\Frame\ANSI UP8 x 30 1771926395577.ipt
- C:\Users\Admin01\Documents\WU15\TRASTRGNN\Inventor\StructureGenerator\Frame\ANSI UP8 x 30 1771926395606.ipt
- C:\Users\Admin01\Documents\WU15\TRASTRGNN\Inventor\StructureGenerator\Frame\ANSI UP8 x 30 1771926395639.ipt
- C:\Users\Admin01\Documents\WU15\TRASTRGNN\Inventor\StructureGenerator\Frame\ANSI UP8 x 30 1771926395668.ipt
- C:\Users\Admin01\Documents\WU15\TRASTRGNN\Inventor\StructureGenerator\Frame\ANSI UP8 x 30 1771926395697.ipt
- C:\Users\Admin01\Documents\WU15\TRASTRGNN\Inventor\StructureGenerator\Frame\ANSI UP8 x 30 1771926395727.ipt
- C:\Users\Admin01\Documents\WU15\TRASTRGNN\Inventor\StructureGenerator\Frame\ANSI UP8 x 30 1771926395757.ipt
- C:\Users\Admin01\Documents\WU15\TRASTRGNN\Inventor\StructureGenerator\Frame\ANSI UP8 x 30 1771926395786.ipt
- C:\Users\Admin01\Documents\WU15\TRASTRGNN\Inventor\StructureGenerator\Frame\ANSI UP8 x 30 1771926395816.ipt
- C:\Users\Admin01\Documents\WU15\TRASTRGNN\Inventor\StructureGenerator\Frame\ANSI UP8 x 30 1771926395845.ipt
- C:\Users\Admin01\Documents\WU15\TRASTRGNN\Inventor\StructureGenerator\Frame\ANSI UP8 x 30 1771926395874.ipt
- C:\Users\Admin01\Documents\WU15\TRASTRGNN\Inventor\StructureGenerator\Frame\ANSI UP8 x 30 1771926395903.ipt
- C:\Users\Admin01\Documents\WU15\TRASTRGNN\Inventor\StructureGenerator\Frame\ANSI UP8 x 30 1771926395932.ipt
- C:\Users\Admin01\Documents\WU15\TRASTRGNN\Inventor\StructureGenerator\Frame\ANSI UP8 x 30 1771926395961.ipt
- C:\Users\Admin01\Documents\WU15\TRASTRGNN\Inventor\StructureGenerator\Frame\ANSI UP8 x 30 1771926395990.ipt
- C:\Users\Admin01\Documents\WU15\TRASTRGNN\Inventor\StructureGenerator\Frame\ANSI UP8 x 30 1771926396020.ipt
- C:\Users\Admin01\Documents\WU15\TRASTRGNN\Inventor\StructureGenerator\Frame\ANSI UP8 x 30 1771926396049.ipt
- C:\Users\Admin01\Documents\WU15\TRASTRGNN\Inventor\StructureGenerator\Frame\ANSI UP8 x 30 1771926396078.ipt
- C:\Users\Admin01\Documents\WU15\TRASTRGNN\Inventor\StructureGenerator\Frame\ANSI UP8 x 30 1771926396107.ipt
- C:\Users\Admin01\Documents\WU15\TRASTRGNN\Inventor\StructureGenerator\Frame\ANSI UP8 x 30 1771926396136.ipt
- C:\Users\Admin01\Documents\WU15\TRASTRGNN\Inventor\StructureGenerator\Frame\ANSI UP8 x 30 1771926396165.ipt
- C:\Users\Admin01\Documents\WU15\TRASTRGNN\Inventor\StructureGenerator\Frame\ANSI UP8 x 30 1771926396195.ipt
- C:\Users\Admin01\Documents\WU15\TRASTRGNN\Inventor\StructureGenerator\Frame\ANSI UP8 x 30 1771926396224.ipt
- C:\Users\Admin01\Documents\WU15\TRASTRGNN\Inventor\StructureGenerator\Frame\ANSI UP8 x 30 1771926396254.ipt
- C:\Users\Admin01\Documents\WU15\TRASTRGNN\Inventor\StructureGenerator\Frame\ANSI UP8 x 30 1771926396283.ipt
- C:\Users\Admin01\Documents\WU15\TRASTRGNN\Inventor\StructureGenerator\Frame\ANSI UP8 x 30 1771926396312.ipt
- C:\Users\Admin01\Documents\WU15\TRASTRGNN\Inventor\StructureGenerator\Frame\ANSI UP8 x 30 1771926396341.ipt
- C:\Users\Admin01\Documents\WU15\TRASTRGNN\Inventor\StructureGenerator\Frame\ANSI UP8 x 30 1771926396370.ipt
- C:\Users\Admin01\Documents\WU15\TRASTRGNN\Inventor\StructureGenerator\Frame\ANSI UP8 x 30 1771926396399.ipt
- C:\Users\Admin01\Documents\WU15\TRASTRGNN\Inventor\StructureGenerator\Frame\ANSI UP8 x 30 1771926396428.ipt
- C:\Users\Admin01\Documents\WU15\TRASTRGNN\Inventor\StructureGenerator\Frame\ANSI UP8 x 30 1771926396458.ipt
- C:\Users\Admin01\Documents\WU15\TRASTRGNN\Inventor\StructureGenerator\Frame\ANSI UP8 x 30 1771926396487.ipt
- C:\Users\Admin01\Documents\WU15\TRASTRGNN\Inventor\StructureGenerator\Frame\ANSI UP8 x 30 1771926396516.ipt
- C:\Users\Admin01\Documents\WU15\TRASTRGNN\Inventor\StructureGenerator\Frame\ANSI UP8 x 30 1771926396545.ipt
- C:\Users\Admin01\Documents\WU15\TRASTRGNN\Inventor\StructureGenerator\Frame\ANSI UP8 x 30 1771926396574.ipt
- C:\Users\Admin01\Documents\WU15\TRASTRGNN\Inventor\StructureGenerator\Frame\ANSI UP8 x 30 1771926396603.ipt
- C:\Users\Admin01\Documents\WU15\TRASTRGNN\Inventor\StructureGenerator\Frame\ANSI UP8 x 30 1771926396633.ipt
- C:\Users\Admin01\Documents\WU15\TRASTRGNN\Inventor\StructureGenerator\Frame\ANSI UP8 x 30 1771926396662.ipt
- C:\Users\Admin01\Documents\WU15\TRASTRGNN\Inventor\StructureGenerator\Frame\ANSI UP8 x 30 1771926396691.ipt
- C:\Users\Admin01\Documents\WU15\TRASTRGNN\Inventor\StructureGenerator\Frame\ANSI UP8 x 30 1771926396722.ipt
- C:\Users\Admin01\Documents\WU15\TRASTRGNN\Inventor\StructureGenerator\Frame\ANSI UP8 x 30 1771926396752.ipt
- C:\Users\Admin01\Documents\WU15\TRASTRGNN\Inventor\StructureGenerator\Frame\ANSI UP8 x 30 1771926396781.ipt
- C:\Users\Admin01\Documents\WU15\TRASTRGNN\Inventor\StructureGenerator\Frame\ANSI UP8 x 30 1771926396810.ipt
- C:\Users\Admin01\Documents\WU15\TRASTRGNN\Inventor\StructureGenerator\Frame\ANSI UP8 x 30 1771926396840.ipt
- C:\Users\Admin01\Documents\WU15\TRASTRGNN\Inventor\StructureGenerator\Frame\ANSI UP8 x 30 1771926396869.ipt
- C:\Users\Admin01\Documents\WU15\TRASTRGNN\Inventor\StructureGenerator\Frame\ANSI UP8 x 30 1771926396899.ipt
- C:\Users\Admin01\Documents\WU15\TRASTRGNN\Inventor\StructureGenerator\Frame\ANSI UP8 x 30 1771926396928.ipt
- C:\Users\Admin01\Documents\WU15\TRASTRGNN\Inventor\StructureGenerator\Frame\ANSI UP8 x 30 1771926396957.ipt
- C:\Users\Admin01\Documents\WU15\TRASTRGNN\Inventor\StructureGenerator\Frame\ANSI UP8 x 30 1771926396986.ipt
- C:\Users\Admin01\Documents\WU15\TRASTRGNN\Inventor\StructureGenerator\Frame\ANSI UP8 x 30 1771926397016.ipt
- C:\Users\Admin01\Documents\WU15\TRASTRGNN\Inventor\StructureGenerator\Frame\ANSI UP8 x 30 1771926397045.ipt
- C:\Users\Admin01\Documents\WU15\TRASTRGNN\Inventor\StructureGenerator\Frame\ANSI UP8 x 30 1771926397074.ipt
- C:\Users\Admin01\Documents\WU15\TRASTRGNN\Inventor\StructureGenerator\Frame\ANSI UP8 x 30 1771926397103.ipt
- C:\Users\Admin01\Documents\WU15\TRASTRGNN\Inventor\StructureGenerator\Frame\ANSI UP8 x 30 1771926397133.ipt
- C:\Users\Admin01\Documents\WU15\TRASTRGNN\Inventor\StructureGenerator\Frame\ANSI UP8 x 30 1771926397162.ipt
- C:\Users\Admin01\Documents\WU15\TRASTRGNN\Inventor\StructureGenerator\Frame\ANSI UP8 x 30 1771926397191.ipt
- C:\Users\Admin01\Documents\WU15\TRASTRGNN\Inventor\StructureGenerator\Frame\ANSI UP8 x 30 1771926397222.ipt
- C:\Users\Admin01\Documents\WU15\TRASTRGNN\Inventor\StructureGenerator\Frame\ANSI UP8 x 30 1771926397251.ipt
- C:\Users\Admin01\Documents\WU15\TRASTRGNN\Inventor\StructureGenerator\Frame\ANSI UP8 x 30 1771926397280.ipt
- C:\Users\Admin01\Documents\WU15\TRASTRGNN\Inventor\StructureGenerator\Frame\ANSI UP8 x 30 1771926397309.ipt
- C:\Users\Admin01\Documents\WU15\TRASTRGNN\Inventor\StructureGenerator\Frame\ANSI UP8 x 30 1771926397339.ipt
- C:\Users\Admin01\Documents\WU15\TRASTRGNN\Inventor\StructureGenerator\Frame\ANSI UP8 x 30 1771926397368.ipt
- C:\Users\Admin01\Documents\WU15\TRASTRGNN\Inventor\StructureGenerator\Frame\ANSI UP8 x 30 1771926397397.ipt
- C:\Users\Admin01\Documents\WU15\TRASTRGNN\Inventor\StructureGenerator\Frame\ANSI UP8 x 30 1771926397426.ipt
- C:\Users\Admin01\Documents\WU15\TRASTRGNN\Inventor\StructureGenerator\Frame\ANSI UP8 x 30 1771926397456.ipt
- C:\Users\Admin01\Documents\WU15\TRASTRGNN\Inventor\StructureGenerator\Frame\ANSI UP8 x 30 1771926397485.ipt
- C:\Users\Admin01\Documents\WU15\TRASTRGNN\Inventor\StructureGenerator\Frame\ANSI UP8 x 30 1771926397514.ipt
- C:\Users\Admin01\Documents\WU15\TRASTRGNN\Inventor\StructureGenerator\Frame\ANSI UP8 x 30 1771926397543.ipt
- C:\Users\Admin01\Documents\WU15\TRASTRGNN\Inventor\StructureGenerator\Frame\ANSI UP8 x 30 1771926397573.ipt
- C:\Users\Admin01\Documents\WU15\TRASTRGNN\Inventor\StructureGenerator\Frame\ANSI UP8 x 30 1771926397602.ipt
- C:\Users\Admin01\Documents\WU15\TRASTRGNN\Inventor\StructureGenerator\Frame\ANSI UP8 x 30 1771926397631.ipt
- C:\Users\Admin01\Documents\WU15\TRASTRGNN\Inventor\StructureGenerator\Frame\ANSI UP8 x 30 1771926397660.ipt
- C:\Users\Admin01\Documents\WU15\TRASTRGNN\Inventor\StructureGenerator\Frame\ANSI UP8 x 30 1771926397689.ipt
- C:\Users\Admin01\Documents\WU15\TRASTRGNN\Inventor\StructureGenerator\Frame\ANSI UP8 x 30 1771926397718.ipt
- C:\Users\Admin01\Documents\WU15\TRASTRGNN\Inventor\StructureGenerator\Frame\ANSI UP8 x 30 1771926397748.ipt
- C:\Users\Admin01\Documents\WU15\TRASTRGNN\Inventor\StructureGenerator\Frame\ANSI UP8 x 30 1771926397777.ipt
- C:\Users\Admin01\Documents\WU15\TRASTRGNN\Inventor\StructureGenerator\Frame\ANSI UP8 x 30 1771926397808.ipt
- C:\Users\Admin01\Documents\WU15\TRASTRGNN\Inventor\StructureGenerator\Frame\ANSI UP8 x 30 1771926397838.ipt
- C:\Users\Admin01\Documents\WU15\TRASTRGNN\Inventor\StructureGenerator\Frame\ANSI UP8 x 30 1771926397867.ipt
- C:\Users\Admin01\Documents\WU15\TRASTRGNN\Inventor\StructureGenerator\Frame\ANSI UP8 x 30 1771926397896.ipt
- C:\Users\Admin01\Documents\WU15\TRASTRGNN\Inventor\StructureGenerator\Frame\ANSI UP8 x 30 1771926397925.ipt
- C:\Users\Admin01\Documents\WU15\TRASTRGNN\Inventor\StructureGenerator\Frame\ANSI UP8 x 30 1771926397955.ipt
- C:\Users\Admin01\Documents\WU15\TRASTRGNN\Inventor\StructureGenerator\Frame\ANSI UP8 x 30 1771926397984.ipt
- C:\Users\Admin01\Documents\WU15\TRASTRGNN\Inventor\StructureGenerator\Frame\ANSI UP8 x 30 1771926398014.ipt
- C:\Users\Admin01\Documents\WU15\TRASTRGNN\Inventor\StructureGenerator\Frame\ANSI UP8 x 30 1771926398043.ipt
- C:\Users\Admin01\Documents\WU15\TRASTRGNN\Inventor\StructureGenerator\Frame\ANSI UP8 x 30 1771926398072.ipt
- C:\Users\Admin01\Documents\WU15\TRASTRGNN\Inventor\StructureGenerator\Frame\ANSI UP8 x 30 1771926398102.ipt
- C:\Users\Admin01\Documents\WU15\TRASTRGNN\Inventor\StructureGenerator\Frame\ANSI UP8 x 30 1771926398131.ipt
- C:\Users\Admin01\Documents\WU15\TRASTRGNN\Inventor\StructureGenerator\Frame\ANSI UP8 x 30 1771926398160.ipt
- C:\Users\Admin01\Documents\WU15\TRASTRGNN\Inventor\StructureGenerator\Frame\ANSI UP8 x 30 1771926398189.ipt
- C:\Users\Admin01\Documents\WU15\TRASTRGNN\Inventor\StructureGenerator\Frame\ANSI UP8 x 30 1771926398218.ipt
- C:\Users\Admin01\Documents\WU15\TRASTRGNN\Inventor\StructureGenerator\Frame\ANSI UP8 x 30 1771926398248.ipt
- C:\Users\Admin01\Documents\WU15\TRASTRGNN\Inventor\StructureGenerator\Frame\ANSI UP8 x 30 1771926398278.ipt
- C:\Users\Admin01\Documents\WU15\TRASTRGNN\Inventor\StructureGenerator\Frame\ANSI UP8 x 30 1771926398307.ipt
- C:\Users\Admin01\Documents\WU15\TRASTRGNN\Inventor\StructureGenerator\Frame\ANSI UP8 x 30 1771926398337.ipt
- C:\Users\Admin01\Documents\WU15\TRASTRGNN\Inventor\StructureGenerator\Frame\ANSI UP8 x 30 1771926398366.ipt
- C:\Users\Admin01\Documents\WU15\TRASTRGNN\Inventor\StructureGenerator\Frame\ANSI UP8 x 30 1771926398395.ipt
- C:\Users\Admin01\Documents\WU15\TRASTRGNN\Inventor\StructureGenerator\Frame\ANSI UP8 x 30 1771926398424.ipt
- C:\Users\Admin01\Documents\WU15\TRASTRGNN\Inventor\StructureGenerator\Frame\ANSI UP8 x 30 1771926398454.ipt
- C:\Users\Admin01\Documents\WU15\TRASTRGNN\Inventor\StructureGenerator\Frame\ANSI UP8 x 30 1771926398483.ipt
- C:\Users\Admin01\Documents\WU15\TRASTRGNN\Inventor\StructureGenerator\Frame\ANSI UP8 x 30 1771926398513.ipt
- C:\Users\Admin01\Documents\WU15\TRASTRGNN\Inventor\StructureGenerator\Frame\ANSI UP8 x 30 1771926398542.ipt
- C:\Users\Admin01\Documents\WU15\TRASTRGNN\Inventor\StructureGenerator\Frame\ANSI UP8 x 30 1771926398571.ipt
- C:\Users\Admin01\Documents\WU15\TRASTRGNN\Inventor\StructureGenerator\Frame\ANSI UP8 x 30 1771926398600.ipt
- C:\Users\Admin01\Documents\WU15\TRASTRGNN\Inventor\StructureGenerator\Frame\ANSI UP8 x 30 1771926398631.ipt
- C:\Users\Admin01\Documents\WU15\TRASTRGNN\Inventor\StructureGenerator\Frame\ANSI UP8 x 30 1771926398660.ipt
- C:\Users\Admin01\Documents\WU15\TRASTRGNN\Inventor\StructureGenerator\Frame\ANSI UP8 x 30 1771926398690.ipt
- C:\Users\Admin01\Documents\WU15\TRASTRGNN\Inventor\StructureGenerator\Frame\ANSI UP8 x 30 1771926398720.ipt
- C:\Users\Admin01\Documents\WU15\TRASTRGNN\Inventor\StructureGenerator\Frame\ANSI UP8 x 30 1771926398749.ipt
- C:\Users\Admin01\Documents\WU15\TRASTRGNN\Inventor\StructureGenerator\Frame\ANSI UP8 x 30 1771926398779.ipt
- C:\Users\Admin01\Documents\WU15\TRASTRGNN\Inventor\StructureGenerator\Frame\ANSI UP8 x 30 1771926398808.ipt
- C:\Users\Admin01\Documents\WU15\TRASTRGNN\Inventor\StructureGenerator\Frame\ANSI UP8 x 30 1771926398837.ipt
- C:\Users\Admin01\Documents\WU15\TRASTRGNN\Inventor\StructureGenerator\Frame\ANSI UP8 x 30 1771926398867.ipt
- C:\Users\Admin01\Documents\WU15\TRASTRGNN\Inventor\StructureGenerator\Frame\ANSI UP8 x 30 1771926398898.ipt
- C:\Users\Admin01\Documents\WU15\TRASTRGNN\Inventor\StructureGenerator\Frame\ANSI UP8 x 30 1771926398928.ipt
- C:\Users\Admin01\Documents\WU15\TRASTRGNN\Inventor\StructureGenerator\Frame\ANSI UP8 x 30 1771926398958.ipt
- C:\Users\Admin01\Documents\WU15\TRASTRGNN\Inventor\StructureGenerator\Frame\ANSI UP8 x 30 1771926398988.ipt
- C:\Users\Admin01\Documents\WU15\TRASTRGNN\Inventor\StructureGenerator\Frame\ANSI UP8 x 30 1771926399018.ipt
- C:\Users\Admin01\Documents\WU15\TRASTRGNN\Inventor\StructureGenerator\Frame\ANSI UP8 x 30 1771926399048.ipt
- C:\Users\Admin01\Documents\WU15\TRASTRGNN\Inventor\StructureGenerator\Frame\ANSI UP8 x 30 1771926399077.ipt
- C:\Users\Admin01\Documents\WU15\TRASTRGNN\Inventor\StructureGenerator\Frame\ANSI UP8 x 30 1771926399106.ipt
- C:\Users\Admin01\Documents\WU15\TRASTRGNN\Inventor\StructureGenerator\Frame\ANSI UP8 x 30 1771926399136.ipt
- C:\Users\Admin01\Documents\WU15\TRASTRGNN\Inventor\StructureGenerator\Frame\ANSI UP8 x 30 1771926399165.ipt
- C:\Users\Admin01\Documents\WU15\TRASTRGNN\Inventor\StructureGenerator\Frame\ANSI UP8 x 30 1771926399195.ipt
- C:\Users\Admin01\Documents\WU15\TRASTRGNN\Inventor\StructureGenerator\Frame\ANSI UP8 x 30 1771926399225.ipt
- C:\Users\Admin01\Documents\WU15\TRASTRGNN\Inventor\StructureGenerator\Frame\ANSI UP8 x 30 1771926399255.ipt
- C:\Users\Admin01\Documents\WU15\TRASTRGNN\Inventor\StructureGenerator\Frame\ANSI UP8 x 30 1771926399285.ipt
- C:\Users\Admin01\Documents\WU15\TRASTRGNN\Inventor\StructureGenerator\Frame\ANSI UP8 x 30 1771926399315.ipt
- C:\Users\Admin01\Documents\WU15\TRASTRGNN\Inventor\StructureGenerator\Frame\ANSI UP8 x 30 1771926399344.ipt
- C:\Users\Admin01\Documents\WU15\TRASTRGNN\Inventor\StructureGenerator\Frame\ANSI UP8 x 30 1771926399374.ipt
- C:\Users\Admin01\Documents\WU15\TRASTRGNN\Inventor\StructureGenerator\Frame\ANSI UP8 x 30 1771926399403.ipt
- C:\Users\Admin01\Documents\WU15\TRASTRGNN\Inventor\StructureGenerator\Frame\ANSI UP8 x 30 1771926399432.ipt
- C:\Users\Admin01\Documents\WU15\TRASTRGNN\Inventor\StructureGenerator\Frame\ANSI UP8 x 30 1771926399462.ipt
- C:\Users\Admin01\Documents\WU15\TRASTRGNN\Inventor\StructureGenerator\Frame\ANSI UP8 x 30 1771926399492.ipt
- C:\Users\Admin01\Documents\WU15\TRASTRGNN\Inventor\StructureGenerator\Frame\ANSI UP8 x 30 1771926399521.ipt
- C:\Users\Admin01\Documents\WU15\TRASTRGNN\Inventor\StructureGenerator\Frame\ANSI UP8 x 30 1771926399551.ipt
- C:\Users\Admin01\Documents\WU15\TRASTRGNN\Inventor\StructureGenerator\Frame\ANSI UP8 x 30 1771926399581.ipt
- C:\Users\Admin01\Documents\WU15\TRASTRGNN\Inventor\StructureGenerator\Frame\ANSI UP8 x 30 1771926399610.ipt
- C:\Users\Admin01\Documents\WU15\TRASTRGNN\Inventor\StructureGenerator\Frame\ANSI UP8 x 30 1771926399640.ipt
- C:\Users\Admin01\Documents\WU15\TRASTRGNN\Inventor\StructureGenerator\Frame\ANSI UP8 x 30 1771926399669.ipt
- C:\Users\Admin01\Documents\WU15\TRASTRGNN\Inventor\StructureGenerator\Frame\ANSI UP8 x 30 1771926399699.ipt
- C:\Users\Admin01\Documents\WU15\TRASTRGNN\Inventor\StructureGenerator\Frame\ANSI UP8 x 30 1771926399730.ipt
- C:\Users\Admin01\Documents\WU15\TRASTRGNN\Inventor\StructureGenerator\Frame\ANSI UP8 x 30 1771926399760.ipt
- C:\Users\Admin01\Documents\WU15\TRASTRGNN\Inventor\StructureGenerator\Frame\ANSI UP8 x 30 1771926399791.ipt
- C:\Users\Admin01\Documents\WU15\TRASTRGNN\Inventor\StructureGenerator\Frame\ANSI UP8 x 30 1771926399820.ipt
- C:\Users\Admin01\Documents\WU15\TRASTRGNN\Inventor\StructureGenerator\Frame\ANSI UP8 x 30 1771926399850.ipt
- C:\Users\Admin01\Documents\WU15\TRASTRGNN\Inventor\StructureGenerator\Frame\ANSI UP8 x 30 1771926399879.ipt
- C:\Users\Admin01\Documents\WU15\TRASTRGNN\Inventor\StructureGenerator\Frame\ANSI UP8 x 30 1771926399909.ipt
- C:\Users\Admin01\Documents\WU15\TRASTRGNN\Inventor\StructureGenerator\Frame\ANSI UP8 x 30 1771926399938.ipt
- C:\Users\Admin01\Documents\WU15\TRASTRGNN\Inventor\StructureGenerator\Frame\ANSI UP8 x 30 1771926399968.ipt
- C:\Users\Admin01\Documents\WU15\TRASTRGNN\Inventor\StructureGenerator\Frame\ANSI UP8 x 30 1771926400000.ipt
- C:\Users\Admin01\Documents\WU15\TRASTRGNN\Inventor\StructureGenerator\Frame\ANSI UP8 x 30 1771926400030.ipt
- C:\Users\Admin01\Documents\WU15\TRASTRGNN\Inventor\StructureGenerator\Frame\ANSI UP8 x 30 1771926400059.ipt
- C:\Users\Admin01\Documents\WU15\TRASTRGNN\Inventor\StructureGenerator\Frame\ANSI UP8 x 30 1771926400089.ipt
- C:\Users\Admin01\Documents\WU15\TRASTRGNN\Inventor\StructureGenerator\Frame\ANSI UP8 x 30 1771926400119.ipt
- C:\Users\Admin01\Documents\WU15\TRASTRGNN\Inventor\StructureGenerator\Frame\ANSI UP8 x 30 1771926400148.ipt